# Autodesk Inventor assembly: Pusher
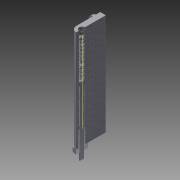
[picture p0: Inventor's stored thumbnail of the model, 180x180]
Saved by Autodesk Inventor 2011 (Build 150239000, 239)
## iProperties
Created: 2011-04-01
Part Number: Pusher
Document SubType Name: Assembly
Designer: Rob
Author: Rob
## Documents named in this file (6)
- C:\Users\M. Woods III\Desktop\design\Mechanical Drawings\pusher_1.iam
- C:\Users\M. Woods III\Desktop\design\Mechanical Drawings\pusher_1_holder.ipt
- C:\Users\M. Woods III\Desktop\design\Mechanical Drawings\pusher_pushrod.ipt
- C:\Users\M. Woods III\Desktop\design\Mechanical Drawings\pusher_springplate.ipt
- C:\Users\M. Woods III\Desktop\design\Mechanical Drawings\pusher_bolt.ipt
- C:\Users\M. Woods III\Desktop\design\Mechanical Drawings\pusher_spring_long.ipt
## Components (9 placed, 5 different names)
1. pusher_1_holder:1 — Mate:1, Mate:2, Mate:4, Mate:12, Mate:13, Mate:14, Mate:17
2. pusher_pushrod:1 — Mate:1, Mate:3, Flush:4
3. pusher_springplate:1 — Mate:2, Mate:15, Flush:2
4. pusher_bolt:1 — Mate:3, Mate:4, Flush:4
5. pusher_springplate:2 — Mate:12, Mate:16, Flush:3
6. pusher_spring_long:1 — Mate:13, Mate:15
7. pusher_spring_long:2 — Mate:14, Flush:2, Mate:16
8. pusher_spring_long:3 — Mate:17, Flush:3, Mate:18, Mate:19
9. pusher_springplate:3 — Mate:18, Mate:19
## Relationships (15: Mate 12, Flush 3)
- Mate:1: pusher_1_holder:1 ↔ pusher_pushrod:1
- Mate:2: pusher_1_holder:1 ↔ pusher_springplate:1
- Mate:3: pusher_pushrod:1 ↔ pusher_bolt:1
- Mate:4: pusher_1_holder:1 ↔ pusher_bolt:1
- Mate:12: pusher_1_holder:1 ↔ pusher_springplate:2
- Mate:13: pusher_1_holder:1 ↔ pusher_spring_long:1
- Mate:14: pusher_1_holder:1 ↔ pusher_spring_long:2
- Mate:15: pusher_springplate:1 ↔ pusher_spring_long:1
- Flush:2: pusher_springplate:1 ↔ pusher_spring_long:2
- Mate:16: pusher_springplate:2 ↔ pusher_spring_long:2
- Mate:17: pusher_1_holder:1 ↔ pusher_spring_long:3
- Flush:3: pusher_springplate:2 ↔ pusher_spring_long:3
- Mate:18: pusher_spring_long:3 ↔ pusher_springplate:3
- Mate:19: pusher_spring_long:3 ↔ pusher_springplate:3
- Flush:4 (-10 mm): pusher_pushrod:1 ↔ pusher_bolt:1
